# Autodesk Inventor assembly: TrackDisplayAssy
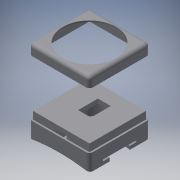
[picture p0: Inventor's stored thumbnail of the model, 180x180]
Saved by Autodesk Inventor 2016 (Build 200138000, 138)
## iProperties
Created: 2016-05-05
Part Number: TrackDisplayAssy
Document SubType Name: Assembly
Designer: xdlea
Author: xdlea
## Documents named in this file (4)
- D:\Library\Documents\7-Git\SPCN-TrackingBracelet\CAD\Version 2\TrackDisplayAssy.iam
- D:\Library\Documents\7-Git\SPCN-TrackingBracelet\CAD\Version 2\TrackDisplayBottom.ipt
- D:\Library\Documents\7-Git\SPCN-TrackingBracelet\CAD\Version 2\TrackDisplayCenter.ipt
- D:\Library\Documents\7-Git\SPCN-TrackingBracelet\CAD\Version 2\TrackDisplayTop.ipt
## Components (3 placed, 3 different names)
1. TrackDisplayBottom:1 — Flush:2, Flush:3, Flush:4, Mate:1
2. TrackDisplayCenter:1 — Flush:4, Mate:1
3. TrackDisplayTop:1 — Flush:2, Flush:3
## Relationships (4: Flush 3, Mate 1)
- Flush:2: TrackDisplayBottom:1 ↔ TrackDisplayTop:1
- Flush:3: TrackDisplayBottom:1 ↔ TrackDisplayTop:1
- Flush:4: TrackDisplayBottom:1 ↔ TrackDisplayCenter:1
- Mate:1: TrackDisplayBottom:1 ↔ TrackDisplayCenter:1
